# Autodesk Inventor assembly: Hand
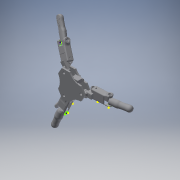
[picture p0: Inventor's stored thumbnail of the model, 180x180]
Saved by Autodesk Inventor 2017 (Build 210142000, 142)
## iProperties
Created: 2016-12-24
Part Number: Hand
Document SubType Name: Assembly
Designer: Samanth
Author: Samanth
## Documents named in this file (6)
- C:\Users\Samanth\Desktop\Purdue Files\Robot\Hand.iam
- C:\Users\Samanth\Desktop\Purdue Files\Robot\Palm1.ipt
- C:\Users\Samanth\Desktop\Purdue Files\Robot\Finger_Joint.ipt
- C:\Users\Samanth\Desktop\Purdue Files\Robot\mainfinger.ipt
- C:\Users\Samanth\Desktop\Purdue Files\Robot\SmallFingerV2.ipt
- C:\Users\Samanth\Desktop\Purdue Files\Robot\Hitec_HS65-MG.ipt
## Components (12 placed, 5 different names)
1. Palm1:1 — Mate:1, Mate:2, Mate:3, Mate:4, Mate:5, Mate:6
2. Finger_Joint:1 — Mate:3, Mate:4, Mate:11, Mate:12, Mate:19
3. Finger_Joint:2 — Mate:5, Mate:6, Mate:9, Mate:10, Mate:20, Mate:21
4. Finger_Joint:3 — Mate:1, Mate:2, Mate:7, Mate:8
5. mainfinger:1 — Mate:7, Mate:8, Mate:13, Mate:14
6. mainfinger:2 — Mate:11, Mate:12, Mate:15, Mate:16
7. mainfinger:3 — Mate:9, Mate:10, Mate:17, Mate:18
8. SmallFingerV2:1 — Mate:15, Mate:16
9. SmallFingerV2:2 — Mate:17, Mate:18
10. SmallFingerV2:3 — Mate:13, Mate:14
11. Palm1:2 — Mate:19, Mate:20, Mate:21
12. Hitec_HS65-MG:1
## Relationships (21: Mate 21)
- Mate:1: Palm1:1 ↔ Finger_Joint:3
- Mate:2: Palm1:1 ↔ Finger_Joint:3
- Mate:3: Palm1:1 ↔ Finger_Joint:1
- Mate:4: Palm1:1 ↔ Finger_Joint:1
- Mate:5: Palm1:1 ↔ Finger_Joint:2
- Mate:6: Palm1:1 ↔ Finger_Joint:2
- Mate:7: Finger_Joint:3 ↔ mainfinger:1
- Mate:8 (-9 mm): Finger_Joint:3 ↔ mainfinger:1
- Mate:9: Finger_Joint:2 ↔ mainfinger:3
- Mate:10 (-9 mm): Finger_Joint:2 ↔ mainfinger:3
- Mate:11: Finger_Joint:1 ↔ mainfinger:2
- Mate:12 (-26 mm): Finger_Joint:1 ↔ mainfinger:2
- Mate:13: mainfinger:1 ↔ SmallFingerV2:3
- Mate:14 (12 mm): mainfinger:1 ↔ SmallFingerV2:3
- Mate:15: mainfinger:2 ↔ SmallFingerV2:1
- Mate:16 (-14 mm): mainfinger:2 ↔ SmallFingerV2:1
- Mate:17: mainfinger:3 ↔ SmallFingerV2:2
- Mate:18 (-16 mm): mainfinger:3 ↔ SmallFingerV2:2
- Mate:19: Finger_Joint:1 ↔ Palm1:2
- Mate:20: Finger_Joint:2 ↔ Palm1:2
- Mate:21: Finger_Joint:2 ↔ Palm1:2
